# Autodesk Inventor assembly: mppcInterface
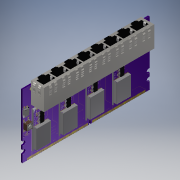
[picture p0: Inventor's stored thumbnail of the model, 180x180]
Saved by Autodesk Inventor 2016 (Build 200138000, 138)
## iProperties
Created: 2016-04-06
Part Number: mppcInterface
Document SubType Name: Assembly
Designer: sawai
Author: sawai
## Documents named in this file (17)
- C:\Users\Jonathan\Documents\Projects\mppcInterface\8-channel\mppcInterface\cad\mppcInterface.iam
- C:\Users\Jonathan\Documents\Projects\mppcInterface\8-channel\mppcInterface\cad\mppcInterfacePcb.ipt
- C:\Users\Jonathan\Documents\Projects\mppcInterface\8-channel\mppcInterface\cad\dependency\mppcHighVoltage\cad\highVoltageMppcBoard.iam
- C:\Users\Jonathan\Documents\Projects\mppcInterface\8-channel\mppcInterface\cad\electronics\32 TQFP.ipt
- C:\Users\Jonathan\Documents\Projects\mppcInterface\8-channel\mppcInterface\cad\electronics\403C.ipt
- C:\Users\Jonathan\Documents\Projects\mppcInterface\8-channel\mppcInterface\cad\electronics\LXDC2HN18A-097.ipt
- C:\Users\Jonathan\Documents\Projects\mppcInterface\8-channel\mppcInterface\cad\electronics\VQFN.ipt
- C:\Users\Jonathan\Documents\Projects\mppcInterface\8-channel\mppcInterface\cad\electronics\QFN-28.ipt
- C:\Users\Jonathan\Documents\Projects\mppcInterface\8-channel\mppcInterface\cad\electronics\soic-8-N.ipt
- C:\Users\Jonathan\Documents\Projects\anodePiShield\coincidenceCounter\cad\electronics\soic\soic.ipt
- C:\Users\Jonathan\Documents\Projects\mppcInterface\8-channel\mppcInterface\cad\electronics\FSM2JSMAA.ipt
- C:\Users\Jonathan\Documents\Projects\mppcInterface\8-channel\mppcInterface\cad\electronics\DX4R005H91.ipt
- C:\Users\Jonathan\Documents\Projects\mppcInterface\8-channel\mppcInterface\cad\connector\SS-668808S-A-PG4-AC.ipt
- C:\Users\Jonathan\Documents\Projects\mppcInterface\8-channel\mppcInterface\cad\electronics\capacitor\capacitor-0402.ipt
- C:\Users\Jonathan\Documents\Projects\mppcInterface\mppcInterface\cad\electronics\capacitor\capacitor.ipt
- C:\Users\Jonathan\Documents\Projects\mppcInterface\8-channel\mppcInterface\cad\electronics\chipResistor\chipResistor-0402.ipt
- C:\Users\Jonathan\Documents\Projects\dynodePiShield\coincidenceCounter\cad\electronics\resistor\chipResistor.ipt
## Components (24 placed, 13 different names)
1. mppcInterfacePcb:1 — Angle:1, Mate:1, Mate:2, Angle:2, Mate:3, Mate:4, Mate:5, Angle:3, Mate:6, Mate:7, Angle:4, Mate:8, Angle:5, Mate:9, Mate:10, Angle:6, Mate:11, Angle:7, Mate:12, Angle:8, Angle:9, Mate:13, Angle:10
2. 32 TQFP:1 — Mate:3
3. 403C:1 — Mate:4
4. LXDC2HN18A-097:1 — Mate:5, Angle:3
5. VQFN:1 — Mate:6, Angle:4
6. QFN-28:1 — Mate:7
7. soic-8-N:1 — Mate:8, Angle:5
8. FSM2JSMAA:1 — Mate:9
9. DX4R005H91:1 — Mate:10, Angle:6
10. SS-668808S-A-PG4-AC:1 — Mate:11, Angle:7
11. capacitor-0402:1 — Flush:1, Mate:12
12. capacitor-0402:2 — Flush:2, Flush:3, Flush:4
13. capacitor-0402:3 — Flush:3, Angle:8
14. capacitor-0402:4 — Flush:4, Angle:9
15. capacitor-0402:5 — Flush:1, Flush:2
16. chipResistor-0402:1 — Mate:13, Angle:10
17. highVoltageMppcBoard:1 [sub-assembly] — Angle:1, Mate:1
18. highVoltageMppcBoard:3 [sub-assembly]
19. highVoltageMppcBoard:4 [sub-assembly]
20. highVoltageMppcBoard:5 [sub-assembly]
21. highVoltageMppcBoard:2 [sub-assembly] — Mate:2, Angle:2
22. highVoltageMppcBoard:6 [sub-assembly]
23. highVoltageMppcBoard:7 [sub-assembly]
24. highVoltageMppcBoard:8 [sub-assembly]
## Component patterns: (4 elements, first: highVoltageMppcBoard:1), (4 elements, first: highVoltageMppcBoard:2)
## Relationships (27: Mate 13, Angle 10, Flush 4)
- Angle:1 (0 deg): mppcInterfacePcb:1 ↔ highVoltageMppcBoard:1
- Mate:1: mppcInterfacePcb:1 ↔ highVoltageMppcBoard:1
- Mate:2: mppcInterfacePcb:1 ↔ highVoltageMppcBoard:2
- Angle:2 (0 deg): mppcInterfacePcb:1 ↔ highVoltageMppcBoard:2
- Mate:3: mppcInterfacePcb:1 ↔ 32 TQFP:1
- Mate:4: mppcInterfacePcb:1 ↔ 403C:1
- Mate:5: mppcInterfacePcb:1 ↔ LXDC2HN18A-097:1
- Angle:3 (0 deg): mppcInterfacePcb:1 ↔ LXDC2HN18A-097:1
- Mate:6: mppcInterfacePcb:1 ↔ VQFN:1
- Mate:7: mppcInterfacePcb:1 ↔ QFN-28:1
- Angle:4 (135 deg): mppcInterfacePcb:1 ↔ VQFN:1
- Mate:8: mppcInterfacePcb:1 ↔ soic-8-N:1
- Angle:5 (0 deg): mppcInterfacePcb:1 ↔ soic-8-N:1
- Mate:9: mppcInterfacePcb:1 ↔ FSM2JSMAA:1
- Mate:10: mppcInterfacePcb:1 ↔ DX4R005H91:1
- Angle:6 (0 deg): mppcInterfacePcb:1 ↔ DX4R005H91:1
- Mate:11: mppcInterfacePcb:1 ↔ SS-668808S-A-PG4-AC:1
- Angle:7 (0 deg): mppcInterfacePcb:1 ↔ SS-668808S-A-PG4-AC:1
- Flush:1: capacitor-0402:1 ↔ capacitor-0402:5
- Flush:2: capacitor-0402:2 ↔ capacitor-0402:5
- Flush:3: capacitor-0402:2 ↔ capacitor-0402:3
- Flush:4: capacitor-0402:2 ↔ capacitor-0402:4
- Mate:12: mppcInterfacePcb:1 ↔ capacitor-0402:1
- Angle:8 (0 deg): mppcInterfacePcb:1 ↔ capacitor-0402:3
- Angle:9 (0 deg): mppcInterfacePcb:1 ↔ capacitor-0402:4
- Mate:13: mppcInterfacePcb:1 ↔ chipResistor-0402:1
- Angle:10 (0 deg): mppcInterfacePcb:1 ↔ chipResistor-0402:1
